# Autodesk Inventor assembly: set2_to_print.-july21iam
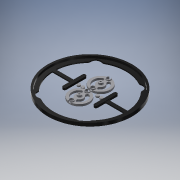
[picture p0: Inventor's stored thumbnail of the model, 180x180]
Saved by Autodesk Inventor 2017 SP1 (Build 210196100, 196)
## iProperties
Created: 2016-07-26
Part Number: set2_to_print.-july21iam
Material: Générique
Document SubType Name: Assembly
Designer: tmonglon
Author: tmonglon
## Documents named in this file (4)
- D:\Inventor\Ahmet\design-files-21jul2017\design-jul2017\design-modified\set2_to_print.-july21iam.iam
- D:\Inventor\Ahmet\mai_2017\modified\bumper_modified2.ipt
- D:\Inventor\Ahmet\design-files-21jul2017\design-jul2017\design\plug_magnet_holder.ipt
- D:\Inventor\Ahmet\design-files-21jul2017\design-jul2017\design-modified\magnet_holder-july21.ipt
## Components (7 placed, 3 different names)
1. bumper_modified2:1 — Placage:1, Placage:2, Affleurement:1, Placage:3, Placage:4, Affleurement:6, Affleurement:7, Placage:7, Placage:8, Placage:9, Placage:10
2. plug_magnet_holder:1 — Affleurement:6, Placage:7, Placage:14
3. plug_magnet_holder:2 — Affleurement:7, Placage:8, Placage:13
4. magnet_holder-july21:1 — Affleurement:2, Placage:4, Placage:9
5. magnet_holder-july21:2 — Affleurement:3, Placage:3, Placage:10
6. plug_magnet_holder:3 — Placage:11, Placage:13
7. plug_magnet_holder:4 — Placage:12, Placage:14
## Relationships (17: Mate 12, Flush 5)
- Placage:1 [Mate]: bumper_modified2:1
- Placage:2 [Mate]: bumper_modified2:1
- Affleurement:1 [Flush]: bumper_modified2:1
- Affleurement:2 [Flush]: magnet_holder-july21:1
- Affleurement:3 [Flush]: magnet_holder-july21:2
- Placage:3 [Mate]: bumper_modified2:1 ↔ magnet_holder-july21:2
- Placage:4 [Mate]: bumper_modified2:1 ↔ magnet_holder-july21:1
- Affleurement:6 [Flush]: bumper_modified2:1 ↔ plug_magnet_holder:1
- Affleurement:7 [Flush]: bumper_modified2:1 ↔ plug_magnet_holder:2
- Placage:7 [Mate]: bumper_modified2:1 ↔ plug_magnet_holder:1
- Placage:8 [Mate]: bumper_modified2:1 ↔ plug_magnet_holder:2
- Placage:9 [Mate] (-16 mm): bumper_modified2:1 ↔ magnet_holder-july21:1
- Placage:10 [Mate] (16 mm): bumper_modified2:1 ↔ magnet_holder-july21:2
- Placage:11 [Mate]: plug_magnet_holder:3
- Placage:12 [Mate]: plug_magnet_holder:4
- Placage:13 [Mate]: plug_magnet_holder:2 ↔ plug_magnet_holder:3
- Placage:14 [Mate]: plug_magnet_holder:1 ↔ plug_magnet_holder:4
